# Autodesk Inventor assembly: Battery
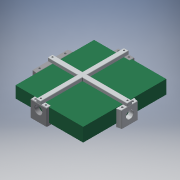
[picture p0: Inventor's stored thumbnail of the model, 180x180]
Saved by Autodesk Inventor 2016 (Build 200138000, 138)
## iProperties
Created: 2015-09-14
Part Number: Battery
Document SubType Name: Assembly
Designer: lachesis
Author: lachesis
## Documents named in this file (5)
- C:\Users\lachesis\git\Swarmie-Build\Swarmie-Assembly\Assemblies\Battery.iam
- C:\Users\lachesis\git\Swarmie-Build\Swarmie-Assembly\Parts\BatteryBase.ipt
- C:\Users\lachesis\git\Swarmie-Build\Swarmie-Assembly\Parts\BatteryInBag.ipt
- C:\Users\lachesis\git\Swarmie-Build\Swarmie-Assembly\Parts\BatteryBrace.ipt
- C:\Users\lachesis\git\Swarmie-Build\Swarmie-Assembly\Parts\BatteryCrossStrap.ipt
## Components (4 placed, 4 different names)
1. BatteryBase:1 — Mate:1, Mate:2, Mate:3, Rigid:2
2. BatteryInBag:1 — Mate:1, Mate:2, Mate:3
3. BatteryBrace:1 — Mate:4
4. BatteryCrossStrap:1 — Rigid:2, Mate:4
## Relationships (5: Mate 4, WeldJoint 1)
- Mate:1: BatteryBase:1 ↔ BatteryInBag:1
- Mate:2: BatteryBase:1 ↔ BatteryInBag:1
- Mate:3: BatteryBase:1 ↔ BatteryInBag:1
- Rigid:2 [WeldJoint]: BatteryBase:1 ↔ BatteryCrossStrap:1
- Mate:4: BatteryBrace:1 ↔ BatteryCrossStrap:1
